# Autodesk Inventor assembly: Structure
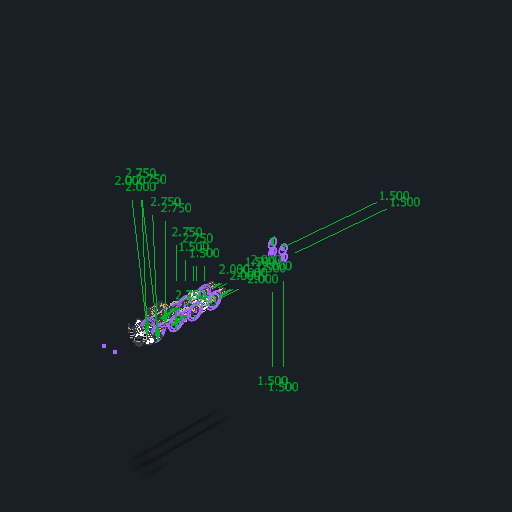
[picture p0: Inventor's stored thumbnail of the model, 512x512]
Saved by Autodesk Inventor 2025.1 (Build 291241000, 241)
## iProperties
Created: 2024-11-04
Part Number: Structure
Document SubType Name: Assembly
Designer: avere
Author: avere
## Documents named in this file (5)
- C:\Users\avere\VEX\High Stakes\CAD\V3\Chassis\Drivebay Right\Structure.iam
- C:\Users\avere\VEX\High Stakes\CAD\V3\Chassis\Drivebay Right\Outer Channel.iam
- C:\Users\avere\VEX\High Stakes\CAD\V3\Chassis\Drivebay Right\Inner Channel.iam
- C:\Users\avere\VEX\High Stakes\CAD\V3\Chassis\Drivebay Right\Knotched Alu C 2x2x2x5.ipt
- C:\Users\avere\VEX\High Stakes\CAD\V3\Chassis\Drivebay Right\MOGO Funnel.iam
## Components (4 placed, 4 different names)
1. Outer Channel:1 [sub-assembly] — Mate:3, Mate:2, Mate:1, Insert:1, Insert:2
2. Inner Channel:1 [sub-assembly] — Mate:3, Mate:2, Mate:1, Mate:4, Mate:5
3. Knotched Alu C 2x2x2x5:1 — Mate:4, Insert:1
4. MOGO Funnel:1 [sub-assembly] — Insert:2, Mate:5
## Relationships (7: Mate 5, Insert 2)
- Mate:3: Outer Channel:1 ↔ Inner Channel:1
- Mate:2: Outer Channel:1 ↔ Inner Channel:1
- Mate:1 (50.8 mm): Outer Channel:1 ↔ Inner Channel:1
- Mate:4: Inner Channel:1 ↔ Knotched Alu C 2x2x2x5:1
- Insert:1: Outer Channel:1 ↔ Knotched Alu C 2x2x2x5:1
- Insert:2: Outer Channel:1 ↔ MOGO Funnel:1
- Mate:5: Inner Channel:1 ↔ MOGO Funnel:1
